# Autodesk Inventor assembly: mesa_0001_00001
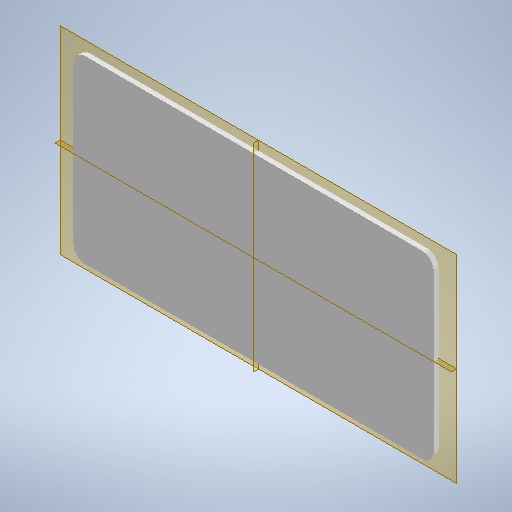
[picture p0: Inventor's stored thumbnail of the model, 512x512]
Saved by Autodesk Inventor 2025.2 (Build 292293000, 293)
## iProperties
Created: 2025-03-28
Part Number: mesa_0001_00001
Document SubType Name: Assembly
Designer: kenne
Author: kenne
## Documents named in this file (2)
- C:\Users\kenne\OneDrive\Ambiente de Trabalho\Robotica & Automação\Sistemas de Microcontroladores\Learning\Inventor\Exercices\Mesa\mesa_0001_00001.iam
- C:\Users\kenne\OneDrive\Ambiente de Trabalho\Robotica & Automação\Sistemas de Microcontroladores\Learning\Inventor\Exercices\Mesa\mesa_0001_00001.ipt
## Components (1 placed, 1 different names)
1. mesa_0001_00001:1 — Flush:1, Flush:2, Flush:3
## Relationships (3: Flush 3)
- Flush:1: mesa_0001_00001:1
- Flush:2: mesa_0001_00001:1
- Flush:3: mesa_0001_00001:1
